# Autodesk Inventor assembly: arm stop 48 degree + switch
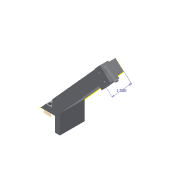
[picture p0: Inventor's stored thumbnail of the model, 180x180]
Saved by Autodesk Inventor 2018 (Build 220112000, 112)
## iProperties
Created: 2019-01-02
Part Number: arm stop 48 degree + switch
Document SubType Name: Assembly
Designer: ball
Author: ball
## Documents named in this file (3)
- C:\FTC\FTC8863CAD\2018Robot\arm stop 48 degree + switch.iam
- C:\FTC\FTC8863CAD\2018Robot\arm stop 48 degree whole.ipt
- C:\FTC\FTC8863CAD\Actobotics\605 parts\605632.ipt
## Components (2 placed, 2 different names)
1. arm stop 48 degree whole:1 — Mate:1, Mate:2, Flush:1
2. 605632:2 — Mate:1, Mate:2, Flush:1
## Relationships (3: Mate 2, Flush 1)
- Mate:1: arm stop 48 degree whole:1 ↔ 605632:2
- Mate:2: arm stop 48 degree whole:1 ↔ 605632:2
- Flush:1: arm stop 48 degree whole:1 ↔ 605632:2
